# Autodesk Inventor assembly: Pinky Finger Assembly
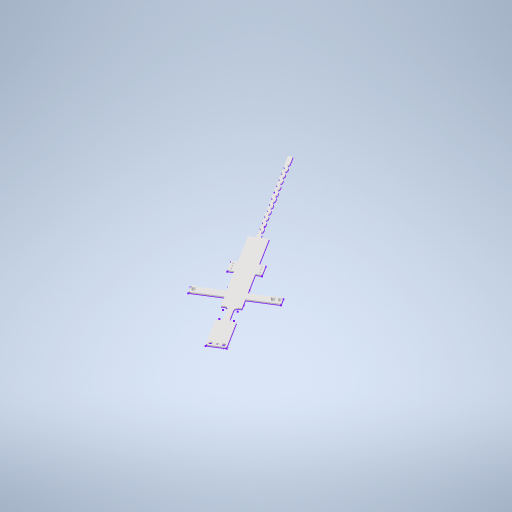
[picture p0: Inventor's stored thumbnail of the model, 512x512]
Saved by Autodesk Inventor 2023.1 (Build 271208000, 208)
## iProperties
Created: 2022-11-29
Part Number: Pinky Finger Assembly
Document SubType Name: Assembly
Designer: petro
Author: petro
## Documents named in this file (4)
- F:\Final Design\Pinky Finger Assembly.iam
- F:\Final Design\Pinky Finger Part.ipt
- F:\Final Design\Medium Peg Part.ipt
- F:\Final Design\Small Peg Part.ipt
## Components (4 placed, 3 different names)
1. Pinky Finger Part:1 — Rotational:1, Rotational:2, Rotational:3
2. Medium Peg Part:1 — Rotational:1
3. Medium Peg Part:2 — Rotational:2
4. Small Peg Part:1 — Rotational:3
## Relationships (3: RevoluteJoint 3)
- Rotational:1 [RevoluteJoint]: Pinky Finger Part:1 ↔ Medium Peg Part:1
- Rotational:2 [RevoluteJoint]: Pinky Finger Part:1 ↔ Medium Peg Part:2
- Rotational:3 [RevoluteJoint]: Pinky Finger Part:1 ↔ Small Peg Part:1
